# Autodesk Inventor assembly: MotorIntake
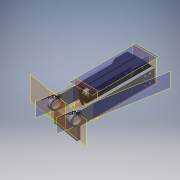
[picture p0: Inventor's stored thumbnail of the model, 180x180]
Saved by Autodesk Inventor 2017 (Build 210142000, 142)
## iProperties
Created: 2017-11-22
Part Number: MotorIntake
Document SubType Name: Assembly
Designer: User
Author: User
## Documents named in this file (4)
- C:\Robotics\CAD\2017-18_CAD\MotorIntake.iam
- C:\Robotics\CAD\2017-18_CAD\WheelIntakeMotorMountTop2.0.ipt
- C:\Robotics\CAD\2017-18_CAD\WheelIntakeMotorMountBottom2.0.ipt
- C:\Robotics\CAD\COTSParts\Rev\REV-41-1300.ipt
## Components (3 placed, 3 different names)
1. WheelIntakeMotorMountTop2.0:1 — Mate:1, Flush:1, Flush:2, Mate:2, Insert:1, Insert:2
2. WheelIntakeMotorMountBottom2.0:1 — Mate:1, Flush:1, Flush:2
3. REV-41-1300:1 — Mate:2, Insert:1, Insert:2
## Relationships (6: Mate 2, Flush 2, Insert 2)
- Mate:1 (35 mm): WheelIntakeMotorMountTop2.0:1 ↔ WheelIntakeMotorMountBottom2.0:1
- Flush:1: WheelIntakeMotorMountTop2.0:1 ↔ WheelIntakeMotorMountBottom2.0:1
- Flush:2: WheelIntakeMotorMountTop2.0:1 ↔ WheelIntakeMotorMountBottom2.0:1
- Mate:2: WheelIntakeMotorMountTop2.0:1 ↔ REV-41-1300:1
- Insert:1: WheelIntakeMotorMountTop2.0:1 ↔ REV-41-1300:1
- Insert:2: WheelIntakeMotorMountTop2.0:1 ↔ REV-41-1300:1
